# Autodesk Inventor assembly: AFL-102-004-01-0C RoadBot Pneumatic Module - AssemblyDrawing
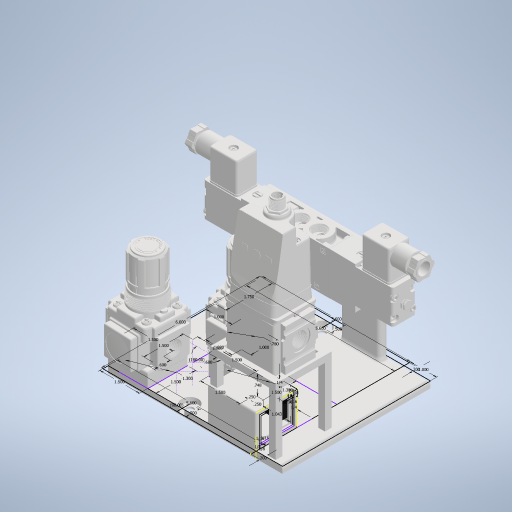
[picture p0: Inventor's stored thumbnail of the model, 512x512]
Saved by Autodesk Inventor 2024.1 (Build 281209000, 209)
## iProperties
Created: 2022-04-02
Part Number: AFL-102-004-01-0C RoadBot Pneumatic Module - AssemblyDrawing
Document SubType Name: Assembly
Designer: Beaucage
Author: Beaucage
## Documents named in this file (6)
- C:\Users\pab2\Documents\GitHub\AFL-hardware-devel\CAD-NewOrgScheme\AFL-102-(TravelAFL)\004-(PneumaticModule)\AFL-102-004-01-0C RoadBot Pneumatic Module - AssemblyDrawing.iam
- C:\Users\pab2\Documents\GitHub\AFL-hardware-devel\CAD-NewOrgScheme\AFL-102-(TravelAFL)\004-(PneumaticModule)\Keystone_Jack_Single_Receptacle (1).ipt
- C:\Users\pab2\Downloads\8812K52_Compressed Air Regulator\8812K52_Compressed Air Regulator.ipt
- C:\Users\pab2\Documents\GitHub\AFL-hardware-devel\CAD-NewOrgScheme\AFL-102-(TravelAFL)\004-(PneumaticModule)\RoadBot Pneumatic Module - Base - r4.ipt
- C:\Users\pab2\Downloads\6425K183_Electrical Air Directional Control Valve\6425K183_Electrical Air Directional Control Valve.ipt
- C:\Users\pab2\Downloads\8083T1_Precision Compressed Air Regulator with Display\8083T1_Precision Compressed Air Regulator with Display.ipt
## Components (6 placed, 5 different names)
1. RoadBot Pneumatic Module - Base - r4:1 — Mate:1, Mate:2, Flush:1, Mate:3, Mate:4, Mate:5, Mate:6, Mate:7, Mate:8, Mate:9, Mate:10, Mate:11, Mate:12, Mate:13
2. Keystone_Jack_Single_Receptacle (1):1 — Mate:1, Mate:2, Flush:1
3. 8812K52_Compressed Air Regulator:1 — Mate:3, Mate:4, Mate:5
4. 8812K52_Compressed Air Regulator:2 — Mate:6, Mate:7
5. 6425K183_Electrical Air Directional Control Valve:1 — Mate:8, Mate:9, Mate:10
6. 8083T1_Precision Compressed Air Regulator with Display:1 — Mate:11, Mate:12, Mate:13
## Relationships (14: Mate 13, Flush 1)
- Mate:1: RoadBot Pneumatic Module - Base - r4:1 ↔ Keystone_Jack_Single_Receptacle (1):1
- Mate:2: RoadBot Pneumatic Module - Base - r4:1 ↔ Keystone_Jack_Single_Receptacle (1):1
- Flush:1: RoadBot Pneumatic Module - Base - r4:1 ↔ Keystone_Jack_Single_Receptacle (1):1
- Mate:3: RoadBot Pneumatic Module - Base - r4:1 ↔ 8812K52_Compressed Air Regulator:1
- Mate:4: RoadBot Pneumatic Module - Base - r4:1 ↔ 8812K52_Compressed Air Regulator:1
- Mate:5: RoadBot Pneumatic Module - Base - r4:1 ↔ 8812K52_Compressed Air Regulator:1
- Mate:6: RoadBot Pneumatic Module - Base - r4:1 ↔ 8812K52_Compressed Air Regulator:2
- Mate:7: RoadBot Pneumatic Module - Base - r4:1 ↔ 8812K52_Compressed Air Regulator:2
- Mate:8: RoadBot Pneumatic Module - Base - r4:1 ↔ 6425K183_Electrical Air Directional Control Valve:1
- Mate:9: RoadBot Pneumatic Module - Base - r4:1 ↔ 6425K183_Electrical Air Directional Control Valve:1
- Mate:10: RoadBot Pneumatic Module - Base - r4:1 ↔ 6425K183_Electrical Air Directional Control Valve:1
- Mate:11: RoadBot Pneumatic Module - Base - r4:1 ↔ 8083T1_Precision Compressed Air Regulator with Display:1
- Mate:12: RoadBot Pneumatic Module - Base - r4:1 ↔ 8083T1_Precision Compressed Air Regulator with Display:1
- Mate:13: RoadBot Pneumatic Module - Base - r4:1 ↔ 8083T1_Precision Compressed Air Regulator with Display:1
